# Autodesk Inventor assembly: J0_Drive
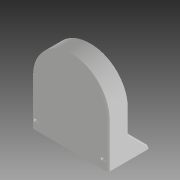
[picture p0: Inventor's stored thumbnail of the model, 180x180]
Saved by Autodesk Inventor 2020 (Build 240168000, 168)
## iProperties
Created: 2021-03-20
Part Number: J0_Drive
Document SubType Name: Assembly
Designer: DDeGo
Author: DDeGo
## Documents named in this file (6)
- C:\Users\DDeGo\Documents\Drew\Projects\OS-ARM\cad\FirstDraft\J1_Drive.iam
- C:\Users\DDeGo\Documents\Drew\Projects\OS-ARM\cad\HarmonicDrive75mm\HarmonicDrive75mm.iam
- C:\Users\DDeGo\Documents\Drew\Projects\OS-ARM\cad\FirstDraft\J1_drivebracket.ipt
- C:\Users\DDeGo\Documents\Drew\Projects\OS-ARM\cad\FirstDraft\J1_motorbracket.ipt
- C:\Users\DDeGo\Documents\Drew\Projects\OS-ARM\cad\OTS\NEMA 23 - 41mm.ipt
- C:\Users\DDeGo\Documents\Drew\Projects\OS-ARM\cad\OTS\6815 bearing.ipt
## Components (5 placed, 5 different names)
1. 6815 bearing:1 — Mate:1, Mate:12, Mate:16, Flush:1
2. HarmonicDrive75mm:1 [sub-assembly] — Mate:12, Mate:15, Mate:16
3. J1_drivebracket:1 — Mate:1, Angle:1, Mate:8, Flush:1
4. J1_motorbracket:1 — Mate:8, Mate:9, Mate:10, Mate:11
5. NEMA 23 - 41mm:1 — Mate:9, Mate:10, Mate:11, Mate:15
## Relationships (10: Mate 8, Angle 1, Flush 1)
- Mate:1: 6815 bearing:1 ↔ J1_drivebracket:1
- Angle:1 (180 deg): J1_drivebracket:1
- Mate:8: J1_drivebracket:1 ↔ J1_motorbracket:1
- Mate:9: J1_motorbracket:1 ↔ NEMA 23 - 41mm:1
- Mate:10: J1_motorbracket:1 ↔ NEMA 23 - 41mm:1
- Mate:11: J1_motorbracket:1 ↔ NEMA 23 - 41mm:1
- Mate:12: 6815 bearing:1 ↔ HarmonicDrive75mm:1
- Mate:15: HarmonicDrive75mm:1 ↔ NEMA 23 - 41mm:1
- Mate:16: 6815 bearing:1 ↔ HarmonicDrive75mm:1
- Flush:1: 6815 bearing:1 ↔ J1_drivebracket:1
